# Autodesk Inventor assembly: 中间轴
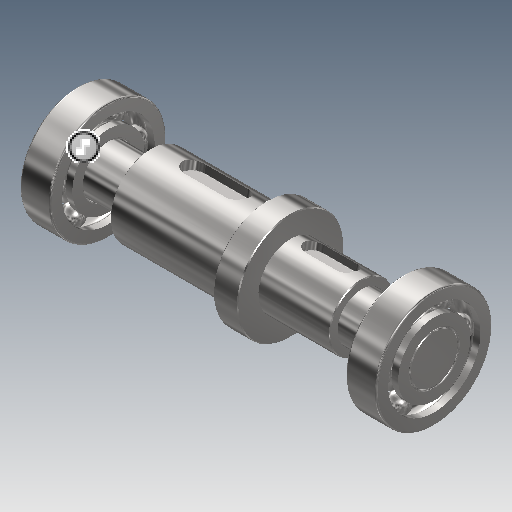
[picture p0: Inventor's stored thumbnail of the model, 512x512]
Saved by Autodesk Inventor 2025 (Build 290162000, 162)
## iProperties
Created: 2025-03-05
Part Number: 中间轴
Document SubType Name: Assembly
Designer: liukan
Author: liukan
## Documents named in this file (4)
- D:\2025春夏那些过往\2025春夏课程文件\机械设计课程设计（甲）\Inventor files\中间轴.iam
- D:\2025春夏那些过往\2025春夏课程文件\机械设计课程设计（甲）\Inventor files\轴2.ipt
- D:\2025春夏那些过往\2025春夏课程文件\机械设计课程设计（甲）\Inventor files\中间轴\设计加速器\轴承1.iam
- D:\2025春夏那些过往\2025春夏课程文件\机械设计课程设计（甲）\Inventor files\中间轴\设计加速器\轴承2.iam
## Components (3 placed, 2 different names)
1. 轴:1 — 配合:1, 配合:2, 表面齐平:1, 表面齐平:2
2. 轴承:1 [sub-assembly] — 配合:1, 表面齐平:2
3. 轴承:2 [sub-assembly] — 配合:2, 表面齐平:1
## Relationships (4: Mate 2, Flush 2)
- 配合:1 [Mate]: 轴:1 ↔ 轴承:1
- 配合:2 [Mate]: 轴:1 ↔ 轴承:2
- 表面齐平:1 [Flush]: 轴:1 ↔ 轴承:2
- 表面齐平:2 [Flush]: 轴:1 ↔ 轴承:1
